# Autodesk Inventor assembly: arm_assembly
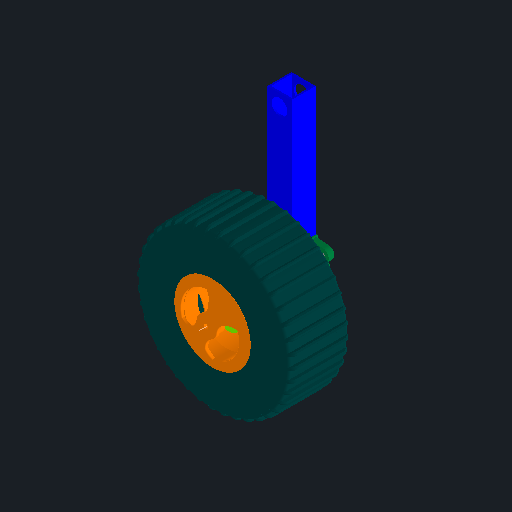
[picture p0: Inventor's stored thumbnail of the model, 512x512]
Saved by Autodesk Inventor 2024 (Build 280153000, 153)
## iProperties
Created: 2023-09-26
Part Number: arm_assembly
Document SubType Name: Assembly
Designer: user
Author: user
## Documents named in this file (4)
- D:\Docs\Robot\3d_v2\machine_body\arm_assembly_l.iam
- D:\Docs\Robot\3d_v2\default_components\motor.ipt
- D:\Docs\Robot\3d_v2\machine_body\arm_assembly\defualt_arm_assembly.iam
- D:\Docs\Robot\3d_v2\machine_body\arm_assembly\wheel_assembly.iam
## Components (3 placed, 3 different names)
1. motor:1 — Вставка:2, Вставка:3
2. defualt_arm_assembly:1 [sub-assembly] — Вставка:2, Совмещение:1, Совмещение:2, Совмещение:3
3. wheel_assembly:1 [sub-assembly] — Вставка:3
## Relationships (5: Mate 3, Insert 2)
- Вставка:2 [Insert]: motor:1 ↔ defualt_arm_assembly:1
- Совмещение:1 [Mate]: defualt_arm_assembly:1
- Совмещение:2 [Mate]: defualt_arm_assembly:1
- Совмещение:3 [Mate]: defualt_arm_assembly:1
- Вставка:3 [Insert]: motor:1 ↔ wheel_assembly:1
